# Autodesk Inventor assembly: Roda Omni 100 mm
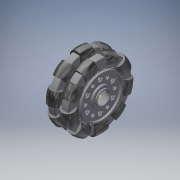
[picture p0: Inventor's stored thumbnail of the model, 180x180]
Saved by Autodesk Inventor 2017.3 (Build 213257000, 257)
## iProperties
Created: 2020-07-21
Part Number: Roda Omni 100 mm
Document SubType Name: Assembly
Designer: Fahar Endra
Author: Fahar Endra
## Documents named in this file (3)
- D:\Robotik KRSBI\Roda Omni 100 mm\Roda Omni 100 mm.iam
- D:\Robotik KRSBI\Roda Omni 100 mm\Dasar.ipt
- D:\Robotik KRSBI\Roda Omni 100 mm\Roller.ipt
## Components (20 placed, 2 different names)
1. Dasar:1 — Rigid:1, Rotational:3, Rotational:4, Rotational:7, Rotational:8, Rotational:14, Rotational:15, Rotational:16, Rotational:17, Rotational:18, Flush:1
2. Dasar:2 — Rigid:1, Rotational:1, Rotational:2, Rotational:5, Rotational:6, Rotational:9, Rotational:10, Rotational:11, Rotational:12, Rotational:13
3. Roller:1 — Rotational:8
4. Roller:2 — Rotational:5
5. Roller:3 — Rotational:4
6. Roller:4 — Rotational:6
7. Roller:5 — Rotational:3
8. Roller:6 — Rotational:7
9. Roller:7 — Rotational:2
10. Roller:8 — Rotational:1
11. Roller:9 — Rotational:9
12. Roller:10 — Rotational:17
13. Roller:11 — Rotational:18
14. Roller:12 — Rotational:12
15. Roller:13 — Rotational:16
16. Roller:14 — Rotational:14
17. Roller:15 — Rotational:15
18. Roller:16 — Rotational:10
19. Roller:17 — Rotational:13
20. Roller:18 — Rotational:11
## Relationships (20: RevoluteJoint 18, WeldJoint 1, Flush 1)
- Rigid:1 [WeldJoint]: Dasar:1 ↔ Dasar:2
- Rotational:1 [RevoluteJoint]: Dasar:2 ↔ Roller:8
- Rotational:2 [RevoluteJoint]: Dasar:2 ↔ Roller:7
- Rotational:3 [RevoluteJoint]: Dasar:1 ↔ Roller:5
- Rotational:4 [RevoluteJoint]: Dasar:1 ↔ Roller:3
- Rotational:5 [RevoluteJoint]: Dasar:2 ↔ Roller:2
- Rotational:6 [RevoluteJoint]: Dasar:2 ↔ Roller:4
- Rotational:7 [RevoluteJoint]: Dasar:1 ↔ Roller:6
- Rotational:8 [RevoluteJoint]: Dasar:1 ↔ Roller:1
- Rotational:9 [RevoluteJoint]: Dasar:2 ↔ Roller:9
- Rotational:10 [RevoluteJoint]: Dasar:2 ↔ Roller:16
- Rotational:11 [RevoluteJoint]: Dasar:2 ↔ Roller:18
- Rotational:12 [RevoluteJoint]: Dasar:2 ↔ Roller:12
- Rotational:13 [RevoluteJoint]: Dasar:2 ↔ Roller:17
- Rotational:14 [RevoluteJoint]: Dasar:1 ↔ Roller:14
- Rotational:15 [RevoluteJoint]: Dasar:1 ↔ Roller:15
- Rotational:16 [RevoluteJoint]: Dasar:1 ↔ Roller:13
- Rotational:17 [RevoluteJoint]: Dasar:1 ↔ Roller:10
- Rotational:18 [RevoluteJoint]: Dasar:1 ↔ Roller:11
- Flush:1 (15.5 mm): Dasar:1
